# Autodesk Inventor assembly: x_axis
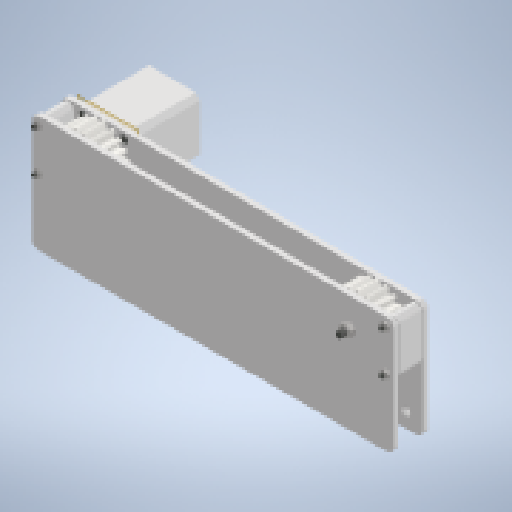
[picture p0: Inventor's stored thumbnail of the model, 512x512]
Saved by Autodesk Inventor 2024 (Build 280153000, 153)
## iProperties
Created: 2026-02-04
Part Number: x_axis
Document SubType Name: Assembly
Designer: SEMEN
Author: SEMEN
## Documents named in this file (14)
- C:\Users\SEMEN\Documents\ETZ2.0\x_axis.iam
- C:\Users\SEMEN\Documents\ETZ2.0\motor_x.ipt
- C:\Users\SEMEN\Documents\ETZ2.0\plate_1.ipt
- C:\Users\SEMEN\Documents\ETZ2.0\x_axis\Design Accelerator\Spur Gears1.iam
- C:\Users\SEMEN\Documents\ETZ2.0\x_axis\Design Accelerator\Spur Gears2.iam
- C:\Users\SEMEN\Documents\Inventor\Content Center Files\R2024\en-US\ISO 7046-1 H(1)\ISO 7046-1 - M3 x 8_ - 4.8 - H - ISO.ipt
- C:\Users\SEMEN\Documents\Inventor\Content Center Files\R2024\en-US\GOST 8338-75\Bearing 23 GOST 8338-75.ipt
- C:\Users\SEMEN\Documents\ETZ2.0\plate_2.ipt
- C:\Users\SEMEN\Documents\Inventor\Content Center Files\R2024\en-US\ISO 7045  H\ISO 7045 - M5 x 35_ - 4.8 - H - ISO.ipt
- C:\Users\SEMEN\Documents\Inventor\Content Center Files\R2024\en-US\ISO 4032(2)\ISO 4032 - M5 - ISO.ipt
- C:\Users\SEMEN\Documents\ETZ2.0\plate_washer_1.ipt
- C:\Users\SEMEN\Documents\Inventor\Content Center Files\R2024\en-US\ISO 7046-1 H(1)\ISO 7046-1 - M3 x 30_ - 4.8 - H - ISO.ipt
- C:\Users\SEMEN\Documents\Inventor\Content Center Files\R2024\en-US\ISO 4032(2)\ISO 4032 - M3 - ISO.ipt
- C:\Users\SEMEN\Documents\ETZ2.0\profile_bearing.ipt
## Components (24 placed, 12 different names)
1. motor_x:1 — Flush:1, Flush:2, Mate:1
2. plate_1:1 — Flush:1, Flush:2, Mate:2, Mate:3, Mate:4, Mate:5, Mate:6, Mate:7, Mate:8, Mate:9, Mate:10, Mate:11, Flush:8, Flush:9, Mate:16, Mate:17, Mate:18, Mate:19, Mate:20, Mate:21, Mate:22, Mate:24, Mate:26, Mate:28, Mate:30, Tangent:1
3. Spur Gears:1 [sub-assembly] — Mate:1, Mate:4
4. Spur Gears:2 [sub-assembly] — Mate:2, Mate:3, Mate:13, Mate:15, Flush:6, Flush:7
5. ISO 7046-1 H M3 x 8 - 4.8 - H:1 — Mate:5
6. ISO 7046-1 H M3 x 8 - 4.8 - H:2 — Mate:6
7. ISO 7046-1 H M3 x 8 - 4.8 - H:3 — Mate:7
8. ISO 7046-1 H M3 x 8 - 4.8 - H:4 — Mate:8
9. plate_2:1 — Flush:5, Mate:12, Mate:23, Mate:25, Mate:27, Mate:29
10. ISO 7045 H M5 x 35 - 4.8 - H:1 — Mate:9, Mate:10
11. ISO 4032 M5:1 — Mate:11, Mate:12
12. Bearing GOST 8338-75 23:1 — Mate:13, Flush:6
13. Bearing GOST 8338-75 23:2 — Mate:15, Flush:7
14. plate_washer_1:1 — Flush:8, Flush:9
15. plate_washer_1:2 — Mate:16, Mate:17
16. ISO 7046-1 H M3 x 30 - 4.8 - H:1 — Mate:18
17. ISO 4032 M3:1 — Mate:22, Mate:23
18. ISO 7046-1 H M3 x 30 - 4.8 - H:2 — Mate:19
19. ISO 7046-1 H M3 x 30 - 4.8 - H:3 — Mate:20
20. ISO 7046-1 H M3 x 30 - 4.8 - H:4 — Mate:21
21. ISO 4032 M3:2 — Mate:24, Mate:25
22. ISO 4032 M3:3 — Mate:26, Mate:27
23. ISO 4032 M3:4 — Mate:28, Mate:29
24. profile_bearing:1 — Mate:30, Tangent:1
## Relationships (37: Mate 29, Flush 7, Tangent 1)
- Flush:1: motor_x:1 ↔ plate_1:1
- Flush:2: motor_x:1 ↔ plate_1:1
- Mate:1: motor_x:1 ↔ Spur Gears:1
- Mate:2: plate_1:1 ↔ Spur Gears:2
- Mate:3 (1 mm): plate_1:1 ↔ Spur Gears:2
- Mate:4 (1 mm): plate_1:1 ↔ Spur Gears:1
- Mate:5: plate_1:1 ↔ ISO 7046-1 H M3 x 8 - 4.8 - H:1
- Mate:6: plate_1:1 ↔ ISO 7046-1 H M3 x 8 - 4.8 - H:2
- Mate:7: plate_1:1 ↔ ISO 7046-1 H M3 x 8 - 4.8 - H:3
- Mate:8: plate_1:1 ↔ ISO 7046-1 H M3 x 8 - 4.8 - H:4
- Flush:5 (22 mm): plate_2:1
- Mate:9: plate_1:1 ↔ ISO 7045 H M5 x 35 - 4.8 - H:1
- Mate:10: plate_1:1 ↔ ISO 7045 H M5 x 35 - 4.8 - H:1
- Mate:11: plate_1:1 ↔ ISO 4032 M5:1
- Mate:12: plate_2:1 ↔ ISO 4032 M5:1
- Mate:13: Spur Gears:2 ↔ Bearing GOST 8338-75 23:1
- Mate:15: Spur Gears:2 ↔ Bearing GOST 8338-75 23:2
- Flush:6: Spur Gears:2 ↔ Bearing GOST 8338-75 23:1
- Flush:7: Spur Gears:2 ↔ Bearing GOST 8338-75 23:2
- Flush:8: plate_1:1 ↔ plate_washer_1:1
- Flush:9: plate_1:1 ↔ plate_washer_1:1
- Mate:16: plate_1:1 ↔ plate_washer_1:2
- Mate:17: plate_1:1 ↔ plate_washer_1:2
- Mate:18: plate_1:1 ↔ ISO 7046-1 H M3 x 30 - 4.8 - H:1
- Mate:19: plate_1:1 ↔ ISO 7046-1 H M3 x 30 - 4.8 - H:2
- Mate:20: plate_1:1 ↔ ISO 7046-1 H M3 x 30 - 4.8 - H:3
- Mate:21: plate_1:1 ↔ ISO 7046-1 H M3 x 30 - 4.8 - H:4
- Mate:22: plate_1:1 ↔ ISO 4032 M3:1
- Mate:23: plate_2:1 ↔ ISO 4032 M3:1
- Mate:24: plate_1:1 ↔ ISO 4032 M3:2
- Mate:25: plate_2:1 ↔ ISO 4032 M3:2
- Mate:26: plate_1:1 ↔ ISO 4032 M3:3
- Mate:27: plate_2:1 ↔ ISO 4032 M3:3
- Mate:28: plate_1:1 ↔ ISO 4032 M3:4
- Mate:29: plate_2:1 ↔ ISO 4032 M3:4
- Mate:30 (0.5 mm): plate_1:1 ↔ profile_bearing:1
- Tangent:1: plate_1:1 ↔ profile_bearing:1
